# Autodesk Inventor assembly: Partical Launcher
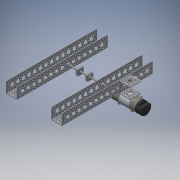
[picture p0: Inventor's stored thumbnail of the model, 180x180]
Saved by Autodesk Inventor 2016 (Build 200138000, 138)
## iProperties
Created: 2016-09-20
Part Number: Partical Launcher
Document SubType Name: Assembly
Designer: Delta
Author: Delta
## Documents named in this file (11)
- C:\Robotics\2016-17_CAD\Partical Launcher.iam
- C:\Robotics\CAD\2015-16\custom cad parts\particle_launcher_Tube.ipt
- C:\Robotics\COTSParts\Tetrix\Tetrix motor_MIR1.ipt
- C:\Robotics\CAD\2015-16\COTSParts\Wheels\Andymark Stealth Wheelam-2648_4inWheel8mmHub (1).iam
- C:\Robotics\COTSParts\Tetrix\Tetrix shaft 250mm.ipt
- C:\Robotics\COTSParts\Tetrix\Tetrix shaft collar.ipt
- C:\Robotics\COTSParts\Actobotics\585 parts\585454.ipt
- C:\Robotics\COTSParts\Actobotics\585 parts\585440.ipt
- C:\Robotics\COTSParts\Actobotics\545 parts\545548.ipt
- C:\Robotics\COTSParts\Actobotics\am-3102NeveRest20 (1).ipt
- C:\Robotics\COTSParts\Actobotics\555 parts\555128.ipt
## Components (18 placed, 10 different names)
1. particle_launcher_Tube:1 — Insert:17, Insert:18
2. Tetrix motor_MIR1:2
3. Andymark Stealth Wheelam-2648_4inWheel8mmHub (1):1 [sub-assembly] — Insert:27
4. Andymark Stealth Wheelam-2648_4inWheel8mmHub (1):2 [sub-assembly] — Insert:28, Insert:29
5. Tetrix shaft 250mm:2 — Insert:35, Insert:36
6. Tetrix shaft collar:1 — Insert:40
7. Tetrix shaft collar:2 — Insert:35, Insert:41
8. Tetrix shaft collar:3 — Insert:39
9. Tetrix shaft collar:4 — Insert:38
10. 585454:1 — Mate:1, Flush:1, Flush:2, Insert:18, Insert:40, Insert:41
11. 585454:2 — Mate:1, Flush:1, Flush:2, Insert:17, Insert:19, Insert:20, Insert:21, Insert:22, Insert:25, Insert:26, Insert:38, Insert:39
12. 585440:2 — Insert:19, Insert:20, Insert:21, Insert:22
13. 545548:1 — Insert:27, Insert:43
14. 545548:2 — Insert:28, Insert:36
15. 545548:3 — Insert:29
16. 555128:1 — Insert:25, Insert:26
17. 555128:2 — Insert:42
18. am-3102NeveRest20 (1):1 — Insert:42, Insert:43
## Relationships (22: Insert 19, Flush 2, Mate 1)
- Mate:1 (114.3 mm): 585454:1 ↔ 585454:2
- Flush:1: 585454:1 ↔ 585454:2
- Flush:2: 585454:1 ↔ 585454:2
- Insert:17: particle_launcher_Tube:1 ↔ 585454:2
- Insert:18: particle_launcher_Tube:1 ↔ 585454:1
- Insert:19: 585454:2 ↔ 585440:2
- Insert:20: 585454:2 ↔ 585440:2
- Insert:21: 585454:2 ↔ 585440:2
- Insert:22: 585454:2 ↔ 585440:2
- Insert:25: 585454:2 ↔ 555128:1
- Insert:26: 585454:2 ↔ 555128:1
- Insert:27: Andymark Stealth Wheelam-2648_4inWheel8mmHub (1):1 ↔ 545548:1
- Insert:28: Andymark Stealth Wheelam-2648_4inWheel8mmHub (1):2 ↔ 545548:2
- Insert:29: Andymark Stealth Wheelam-2648_4inWheel8mmHub (1):2 ↔ 545548:3
- Insert:35 (-137.16 mm): Tetrix shaft 250mm:2 ↔ Tetrix shaft collar:2
- Insert:36 (-96.266 mm): Tetrix shaft 250mm:2 ↔ 545548:2
- Insert:38: Tetrix shaft collar:4 ↔ 585454:2
- Insert:39: Tetrix shaft collar:3 ↔ 585454:2
- Insert:40: Tetrix shaft collar:1 ↔ 585454:1
- Insert:41: Tetrix shaft collar:2 ↔ 585454:1
- Insert:42: 555128:2 ↔ am-3102NeveRest20 (1):1
- Insert:43: 545548:1 ↔ am-3102NeveRest20 (1):1
